# Autodesk Inventor assembly: Joes_Robot
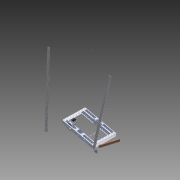
[picture p0: Inventor's stored thumbnail of the model, 180x180]
Saved by Autodesk Inventor 2015 SP1 (Build 190203100, 203)
## iProperties
Created: 2015-01-23
Part Number: Joes_Robot
Document SubType Name: Assembly
Designer: 55221
Author: 55221
## Documents named in this file (20)
- Z:\RoboEaglesCAD\2015CAD\Misc\Joes_Robot.iam
- Z:\RoboEaglesCAD\2015CAD\wheelBase\Outside Sheet Square.ipt
- Z:\RoboEaglesCAD\2015CAD\wheelBase\2x3 Hole Bracket.ipt
- Z:\RoboEaglesCAD\2015CAD\wheelBase\Inside Sheet Square.ipt
- Z:\RoboEaglesCAD\2015CAD\Motion\GuidanceShaft.ipt
- Z:\RoboEaglesCAD\2015CAD\Motion\Roller.ipt
- Z:\RoboEaglesCAD\2015CAD\wheelBase\churroLong.ipt
- Z:\RoboEaglesCAD\2015CAD\wheelBase\TB Output Shaft Hex L-Base 2.ipt
- Z:\RoboEaglesCAD\2015CAD\wheelBase\GBBearing.ipt
- Z:\RoboEaglesCAD\2015CAD\wheelBase\CIM Motor SW.ipt
- Z:\RoboEaglesCAD\2015CAD\wheelBase\gearBoxSimple\simpleGBHousing.ipt
- Z:\RoboEaglesCAD\2015CAD\wheelBase\gearBoxSimple\simpleGBMount.ipt
- Z:\RoboEaglesCAD\2015CAD\wheelBase\gearBoxSimple\simpleGBStopBlockSmallCylindrical.ipt
- Z:\RoboEaglesCAD\2015CAD\Misc\Crossbar.ipt
- Z:\RoboEaglesCAD\2015CAD\Motion\pneumaticHub.ipt
- Z:\RoboEaglesCAD\2015CAD\Motion\pneumaticTyre.ipt
- Z:\RoboEaglesCAD\2015CAD\Misc\Imported Components\90framing\90framing.ipt
- Z:\RoboEaglesCAD\2015CAD\Misc\Imported Components\specialScrews\specialScrews.ipt
- Z:\RoboEaglesCAD\2015CAD\Misc\Imported Components\verticalEndCaps\verticalEndCaps.ipt
- Z:\RoboEaglesCAD\2015CAD\actualWheelBase\Drive Base\Parts\Imported Components\AM14U2 Half Long.iam\Sheet Metal Front-Back.ipt
## Components (29 placed, 20 different names)
1. Outside Sheet Square:1 — Mate:122, Mate:123, Mate:124, Mate:175, Mate:176
2. 2x3 Hole Bracket:1 — Mate:119, Mate:120, Mate:121, Mate:122, Mate:123
3. 2x3 Hole Bracket:2 — Mate:116, Mate:117, Mate:118, Mate:124
4. Inside Sheet Square:1 — Mate:116, Mate:117, Mate:118, Mate:119, Mate:120, Mate:121, Mate:149, Mate:150, Mate:174, Mate:177
5. Inside Sheet Square:2 — Mate:131, Mate:132, Mate:134, Mate:136, Mate:137, Mate:166, Mate:168, Mate:169, Mate:172, Mate:173
6. Outside Sheet Square:2 — Mate:133, Mate:135, Mate:138, Mate:164, Mate:165, Mate:167, Mate:170, Mate:171
7. 2x3 Hole Bracket:3 — Mate:131, Mate:132, Mate:133, Mate:134
8. 2x3 Hole Bracket:4 — Mate:135, Mate:136, Mate:137, Mate:138
9. GuidanceShaft:1 — Angle:4, Mate:145, Mate:146, Mate:153, Mate:154, Mate:155, Angle:8, Mate:157, Mate:158, Mate:160, Mate:161
10. GuidanceShaft:2
11. Roller:1 — Angle:4, Mate:145, Mate:146
12. churroLong:2
13. GBBearing:2
14. CIM Motor SW:3 — Mate:111, Mate:112
15. simpleGBHousing:1 — Mate:102, Mate:103, Mate:104, Mate:105, Mate:106, Mate:111, Mate:112, Mate:149
16. simpleGBMount:1 — Mate:102, Mate:103, Mate:104
17. TB Output Shaft Hex L-Base 2:3 — Mate:108, Mate:150, Mate:151, Mate:152
18. simpleGBStopBlockSmallCylindrical:1 — Mate:105, Mate:106, Mate:108, Mate:151
19. Crossbar:1
20. pneumaticHub:1 — Insert:1, Angle:6, Mate:152
21. pneumaticHub:2 — Insert:1, Insert:2, Angle:6
22. pneumaticTyre:1 — Insert:2
23. 90framing:1
24. 90framing:2 — Mate:159, Mate:162, Mate:163
25. specialScrews:1 — Mate:160, Mate:161, Mate:162, Mate:163
26. verticalEndCaps:1 — Mate:153, Mate:154, Mate:155
27. specialScrews:2 — Angle:8, Mate:157, Mate:158, Mate:159
28. Sheet Metal Front-Back_19 — Mate:164, Mate:165, Mate:166, Mate:167, Mate:168
29. Sheet Metal Front-Back:2 — Mate:169, Mate:170, Mate:171, Mate:172, Mate:173, Mate:174, Mate:175, Mate:176, Mate:177
## Relationships (60: Mate 55, Angle 3, Insert 2)
- Mate:102: simpleGBHousing:1 ↔ simpleGBMount:1
- Mate:103: simpleGBHousing:1 ↔ simpleGBMount:1
- Mate:104: simpleGBHousing:1 ↔ simpleGBMount:1
- Mate:105: simpleGBHousing:1 ↔ simpleGBStopBlockSmallCylindrical:1
- Mate:106: simpleGBHousing:1 ↔ simpleGBStopBlockSmallCylindrical:1
- Mate:108: TB Output Shaft Hex L-Base 2:3 ↔ simpleGBStopBlockSmallCylindrical:1
- Mate:111: CIM Motor SW:3 ↔ simpleGBHousing:1
- Mate:112: CIM Motor SW:3 ↔ simpleGBHousing:1
- Mate:116: 2x3 Hole Bracket:2 ↔ Inside Sheet Square:1
- Mate:117: 2x3 Hole Bracket:2 ↔ Inside Sheet Square:1
- Mate:118: 2x3 Hole Bracket:2 ↔ Inside Sheet Square:1
- Mate:119: 2x3 Hole Bracket:1 ↔ Inside Sheet Square:1
- Mate:120: 2x3 Hole Bracket:1 ↔ Inside Sheet Square:1
- Mate:121: 2x3 Hole Bracket:1 ↔ Inside Sheet Square:1
- Mate:122: Outside Sheet Square:1 ↔ 2x3 Hole Bracket:1
- Mate:123: Outside Sheet Square:1 ↔ 2x3 Hole Bracket:1
- Mate:124: Outside Sheet Square:1 ↔ 2x3 Hole Bracket:2
- Mate:131: Inside Sheet Square:2 ↔ 2x3 Hole Bracket:3
- Mate:132: Inside Sheet Square:2 ↔ 2x3 Hole Bracket:3
- Mate:133: Outside Sheet Square:2 ↔ 2x3 Hole Bracket:3
- Mate:134: Inside Sheet Square:2 ↔ 2x3 Hole Bracket:3
- Mate:135: Outside Sheet Square:2 ↔ 2x3 Hole Bracket:4
- Mate:136: Inside Sheet Square:2 ↔ 2x3 Hole Bracket:4
- Mate:137: Inside Sheet Square:2 ↔ 2x3 Hole Bracket:4
- Mate:138: Outside Sheet Square:2 ↔ 2x3 Hole Bracket:4
- Angle:4 (0 deg): GuidanceShaft:1 ↔ Roller:1
- Mate:145 (22.86 mm): GuidanceShaft:1 ↔ Roller:1
- Mate:146 (3.302 mm): GuidanceShaft:1 ↔ Roller:1
- Mate:149: Inside Sheet Square:1 ↔ simpleGBHousing:1
- Mate:150: Inside Sheet Square:1 ↔ TB Output Shaft Hex L-Base 2:3
- Mate:151: TB Output Shaft Hex L-Base 2:3 ↔ simpleGBStopBlockSmallCylindrical:1
- Insert:1: pneumaticHub:1 ↔ pneumaticHub:2
- Insert:2 (38.1 mm): pneumaticHub:2 ↔ pneumaticTyre:1
- Angle:6 (0 deg): pneumaticHub:1 ↔ pneumaticHub:2
- Mate:152: TB Output Shaft Hex L-Base 2:3 ↔ pneumaticHub:1
- Mate:153: GuidanceShaft:1 ↔ verticalEndCaps:1
- Mate:154: GuidanceShaft:1 ↔ verticalEndCaps:1
- Mate:155: GuidanceShaft:1 ↔ verticalEndCaps:1
- Angle:8 (0 deg): GuidanceShaft:1 ↔ specialScrews:2
- Mate:157: GuidanceShaft:1 ↔ specialScrews:2
- Mate:158 (1.016 mm): GuidanceShaft:1 ↔ specialScrews:2
- Mate:159: 90framing:2 ↔ specialScrews:2
- Mate:160: GuidanceShaft:1 ↔ specialScrews:1
- Mate:161 (-18.288 mm): GuidanceShaft:1 ↔ specialScrews:1
- Mate:162: 90framing:2 ↔ specialScrews:1
- Mate:163: 90framing:2 ↔ specialScrews:1
- Mate:164: Outside Sheet Square:2 ↔ Sheet Metal Front-Back_19
- Mate:165: Outside Sheet Square:2 ↔ Sheet Metal Front-Back_19
- Mate:166: Inside Sheet Square:2 ↔ Sheet Metal Front-Back_19
- Mate:167: Outside Sheet Square:2 ↔ Sheet Metal Front-Back_19
- Mate:168: Inside Sheet Square:2 ↔ Sheet Metal Front-Back_19
- Mate:169: Inside Sheet Square:2 ↔ Sheet Metal Front-Back:2
- Mate:170: Outside Sheet Square:2 ↔ Sheet Metal Front-Back:2
- Mate:171: Outside Sheet Square:2 ↔ Sheet Metal Front-Back:2
- Mate:172: Inside Sheet Square:2 ↔ Sheet Metal Front-Back:2
- Mate:173: Inside Sheet Square:2 ↔ Sheet Metal Front-Back:2
- Mate:174: Inside Sheet Square:1 ↔ Sheet Metal Front-Back:2
- Mate:175: Outside Sheet Square:1 ↔ Sheet Metal Front-Back:2
- Mate:176: Outside Sheet Square:1 ↔ Sheet Metal Front-Back:2
- Mate:177: Inside Sheet Square:1 ↔ Sheet Metal Front-Back:2
